# Autodesk Inventor assembly: Water Table
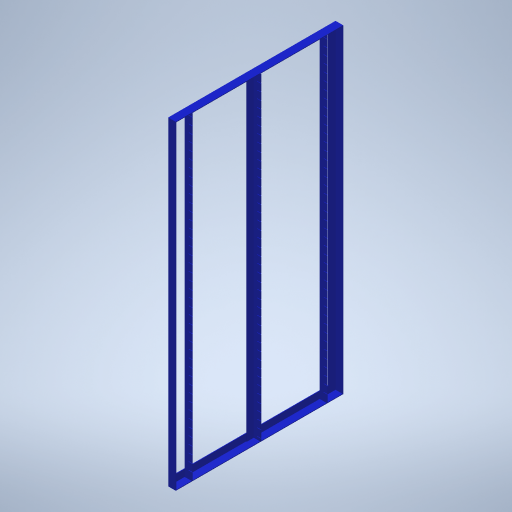
[picture p0: Inventor's stored thumbnail of the model, 512x512]
Saved by Autodesk Inventor 2024.2 (Build 282272000, 272)
## iProperties
Created: 2017-12-18
Part Number: Water Table
Document SubType Name: Assembly
Designer: torba
Author: torba
## Documents named in this file (6)
- D:\GIT\TP_Plasma-Board\CAD\Plasma 5x10\Water Table.iam
- D:\GIT\TP_Plasma-Board\CAD\Plasma 5x10\3 x 3 angle 45 .25 steel\3 x 3 angle 45 .25 steel-66.ipt
- C:\Users\torba\OneDrive\Documents\Inventor\Plasma 5x10\3 x 3 angle 45 .25 steel.ipt
- D:\GIT\TP_Plasma-Board\CAD\Plasma 5x10\3 x 3 angle 45 .25 steel\3 x 3 angle 45 .25 steel-126.ipt
- D:\GIT\TP_Plasma-Board\CAD\Plasma 5x10\1-16 sheet metal.ipt
- D:\GIT\TP_Plasma-Board\CAD\Plasma 5x10\3 x 3.25 steel side slit for 5x10.ipt
## Components (8 placed, 4 different names)
1. 3 x 3 angle 45 .25 steel-126:1 — Flush:2, Mate:3, Mate:4, Flush:3, Mate:6, Mate:10, Mate:16, Mate:18
2. 3 x 3 angle 45 .25 steel-126:2 — Mate:1, Flush:1, Mate:2, Mate:5, Mate:7, Mate:8, Mate:17
3. 3 x 3 angle 45 .25 steel-66:3 — Mate:1, Flush:1, Mate:2, Flush:2, Mate:3, Mate:4, Mate:9, Mate:11, Mate:12, Mate:15
4. 3 x 3 angle 45 .25 steel-66:4 — Flush:3, Mate:5, Mate:6, Mate:13, Mate:14
5. 1-16 sheet metal:1 — Mate:7, Mate:8, Mate:9
6. 3 x 3.25 steel side slit for 5x10:1 — Mate:11, Mate:15, Mate:18
7. 3 x 3.25 steel side slit for 5x10:2 — Mate:12, Mate:14, Mate:17
8. 3 x 3.25 steel side slit for 5x10:3 — Mate:10, Mate:13, Mate:16
## Relationships (21: Mate 18, Flush 3)
- Mate:1: 3 x 3 angle 45 .25 steel-126:2 ↔ 3 x 3 angle 45 .25 steel-66:3
- Flush:1: 3 x 3 angle 45 .25 steel-126:2 ↔ 3 x 3 angle 45 .25 steel-66:3
- Mate:2: 3 x 3 angle 45 .25 steel-126:2 ↔ 3 x 3 angle 45 .25 steel-66:3
- Flush:2: 3 x 3 angle 45 .25 steel-126:1 ↔ 3 x 3 angle 45 .25 steel-66:3
- Mate:3: 3 x 3 angle 45 .25 steel-126:1 ↔ 3 x 3 angle 45 .25 steel-66:3
- Mate:4: 3 x 3 angle 45 .25 steel-126:1 ↔ 3 x 3 angle 45 .25 steel-66:3
- Flush:3: 3 x 3 angle 45 .25 steel-126:1 ↔ 3 x 3 angle 45 .25 steel-66:4
- Mate:5: 3 x 3 angle 45 .25 steel-126:2 ↔ 3 x 3 angle 45 .25 steel-66:4
- Mate:6: 3 x 3 angle 45 .25 steel-126:1 ↔ 3 x 3 angle 45 .25 steel-66:4
- Mate:7: 3 x 3 angle 45 .25 steel-126:2 ↔ 1-16 sheet metal:1
- Mate:8: 3 x 3 angle 45 .25 steel-126:2 ↔ 1-16 sheet metal:1
- Mate:9: 3 x 3 angle 45 .25 steel-66:3 ↔ 1-16 sheet metal:1
- Mate:10: 3 x 3 angle 45 .25 steel-126:1 ↔ 3 x 3.25 steel side slit for 5x10:3
- Mate:11: 3 x 3 angle 45 .25 steel-66:3 ↔ 3 x 3.25 steel side slit for 5x10:1
- Mate:12: 3 x 3 angle 45 .25 steel-66:3 ↔ 3 x 3.25 steel side slit for 5x10:2
- Mate:13: 3 x 3 angle 45 .25 steel-66:4 ↔ 3 x 3.25 steel side slit for 5x10:3
- Mate:14: 3 x 3 angle 45 .25 steel-66:4 ↔ 3 x 3.25 steel side slit for 5x10:2
- Mate:15: 3 x 3 angle 45 .25 steel-66:3 ↔ 3 x 3.25 steel side slit for 5x10:1
- Mate:16 (152.4 mm): 3 x 3 angle 45 .25 steel-126:1 ↔ 3 x 3.25 steel side slit for 5x10:3
- Mate:17 (152.4 mm): 3 x 3 angle 45 .25 steel-126:2 ↔ 3 x 3.25 steel side slit for 5x10:2
- Mate:18 (838.2 mm): 3 x 3 angle 45 .25 steel-126:1 ↔ 3 x 3.25 steel side slit for 5x10:1
